# Autodesk Inventor assembly: Battery_18650_asembly
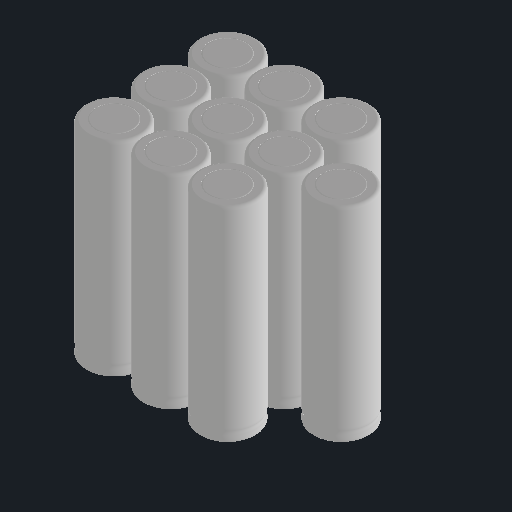
[picture p0: Inventor's stored thumbnail of the model, 512x512]
Saved by Autodesk Inventor 2024 (Build 280153000, 153)
## iProperties
Created: 2023-05-15
Part Number: Battery_18650_asembly
Document SubType Name: Assembly
Designer: user
Author: user
## Documents named in this file (2)
- D:\Docs\Robot\3d_v2\electronics\Battery_18650_asembly.iam
- D:\Docs\Robot\3d_v2\electronics\Battery_18650.ipt
## Components (10 placed, 1 different names)
1. Battery_18650:1 — Совмещение:1, Совмещение:2, Совмещение:3, Заподлицо:1, Касательность:1, Заподлицо:2, Касательность:3, Совмещение:4
2. Battery_18650:2 — Заподлицо:1, Касательность:1, Касательность:2, Совмещение:4, Совмещение:5, Касательность:5, Совмещение:7
3. Battery_18650:3 — Заподлицо:2, Заподлицо:3, Касательность:3, Касательность:4, Совмещение:6, Касательность:12
4. Battery_18650:4 — Заподлицо:3, Касательность:2, Касательность:4, Совмещение:5, Совмещение:6, Заподлицо:4, Заподлицо:5, Касательность:7, Касательность:11, Совмещение:8
5. Battery_18650:5 — Заподлицо:5, Касательность:5, Касательность:6, Совмещение:7
6. Battery_18650:6 — Заподлицо:4, Касательность:6, Касательность:7, Заподлицо:6, Касательность:10, Совмещение:9
7. Battery_18650:7 — Заподлицо:6, Заподлицо:7, Касательность:8, Касательность:12, Совмещение:11
8. Battery_18650:8 — Заподлицо:8, Касательность:9, Касательность:10, Совмещение:9, Совмещение:10
9. Battery_18650:9 — Заподлицо:7, Заподлицо:8, Касательность:8, Касательность:9, Касательность:11, Совмещение:8, Совмещение:10, Совмещение:11, Заподлицо:9, Касательность:13, Совмещение:12
10. Battery_18650:10 — Заподлицо:9, Касательность:13, Совмещение:12
## Relationships (34: Tangent 13, Mate 12, Flush 9)
- Совмещение:1 [Mate]: Battery_18650:1
- Совмещение:2 [Mate]: Battery_18650:1
- Совмещение:3 [Mate]: Battery_18650:1
- Заподлицо:1 [Flush]: Battery_18650:1 ↔ Battery_18650:2
- Касательность:1 [Tangent]: Battery_18650:1 ↔ Battery_18650:2
- Заподлицо:2 [Flush]: Battery_18650:1 ↔ Battery_18650:3
- Заподлицо:3 [Flush]: Battery_18650:3 ↔ Battery_18650:4
- Касательность:2 [Tangent]: Battery_18650:2 ↔ Battery_18650:4
- Касательность:3 [Tangent]: Battery_18650:1 ↔ Battery_18650:3
- Касательность:4 [Tangent]: Battery_18650:3 ↔ Battery_18650:4
- Совмещение:4 [Mate]: Battery_18650:1 ↔ Battery_18650:2
- Совмещение:5 [Mate]: Battery_18650:2 ↔ Battery_18650:4
- Совмещение:6 [Mate]: Battery_18650:3 ↔ Battery_18650:4
- Заподлицо:4 [Flush]: Battery_18650:4 ↔ Battery_18650:6
- Заподлицо:5 [Flush]: Battery_18650:4 ↔ Battery_18650:5
- Касательность:5 [Tangent]: Battery_18650:2 ↔ Battery_18650:5
- Касательность:6 [Tangent]: Battery_18650:5 ↔ Battery_18650:6
- Касательность:7 [Tangent]: Battery_18650:4 ↔ Battery_18650:6
- Совмещение:7 [Mate]: Battery_18650:2 ↔ Battery_18650:5
- Заподлицо:6 [Flush]: Battery_18650:6 ↔ Battery_18650:7
- Заподлицо:7 [Flush]: Battery_18650:7 ↔ Battery_18650:9
- Заподлицо:8 [Flush]: Battery_18650:8 ↔ Battery_18650:9
- Касательность:8 [Tangent]: Battery_18650:7 ↔ Battery_18650:9
- Касательность:9 [Tangent]: Battery_18650:8 ↔ Battery_18650:9
- Касательность:10 [Tangent]: Battery_18650:6 ↔ Battery_18650:8
- Касательность:11 [Tangent]: Battery_18650:4 ↔ Battery_18650:9
- Касательность:12 [Tangent]: Battery_18650:3 ↔ Battery_18650:7
- Совмещение:8 [Mate]: Battery_18650:4 ↔ Battery_18650:9
- Совмещение:9 [Mate]: Battery_18650:6 ↔ Battery_18650:8
- Совмещение:10 [Mate]: Battery_18650:8 ↔ Battery_18650:9
- Совмещение:11 [Mate]: Battery_18650:7 ↔ Battery_18650:9
- Заподлицо:9 [Flush]: Battery_18650:9 ↔ Battery_18650:10
- Касательность:13 [Tangent]: Battery_18650:9 ↔ Battery_18650:10
- Совмещение:12 [Mate]: Battery_18650:9 ↔ Battery_18650:10
